# Autodesk Inventor assembly: LeftMecanumDTANewAttachment
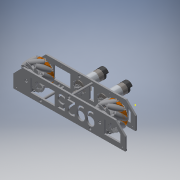
[picture p0: Inventor's stored thumbnail of the model, 180x180]
Saved by Autodesk Inventor 2017 (Build 210142000, 142)
## iProperties
Created: 2017-08-12
Part Number: LeftMecanumDTANewAttachment
Document SubType Name: Assembly
Designer: User
Author: User
## Documents named in this file (7)
- C:\Robotics\CAD\2016-17_CAD\DriveTrain\LeftMecanumDTANewAttachment.iam
- C:\Robotics\CAD\2016-17_CAD\DriveTrain\DrainTrainPlate2.0LeftOutside.iam
- C:\Robotics\CAD\2016-17_CAD\DriveTrain\DriveTrainPlate2.0LeftInside.ipt
- C:\Robotics\CAD\2016-17_CAD\DriveTrain\wheel sub assembly mechanum wheels .iam
- C:\Robotics\CAD\2016-17_CAD\DriveTrain\motor sub assembley.iam
- C:\Robotics\CAD\COTSParts\Tetrix\tetrix-motor-mounts-1.snapshot.1\Tetrex 2pc motor mount.ipt
- C:\Robotics\CAD\2016-17_CAD\DriveTrain\drive train standoff.0002.ipt
## Components (11 placed, 6 different names)
1. DrainTrainPlate2.0LeftOutside:1 [sub-assembly] — Flush:2, Mate:3, Flush:3, Mate:4, Flush:5, Mate:14, Mate:15, Mate:16
2. DriveTrainPlate2.0LeftInside:1 — Mate:2, Flush:4, Mate:5, Flush:6, Mate:6, Mate:7, Mate:8, Mate:10, Mate:11, Mate:12
3. wheel sub assembly mechanum wheels :1 [sub-assembly] — Mate:4, Flush:5, Mate:5, Flush:6, Flush:7
4. wheel sub assembly mechanum wheels :2 [sub-assembly] — Flush:2, Mate:2, Mate:3, Flush:3, Flush:4, Flush:8
5. motor sub assembley:1 [sub-assembly] — Mate:13, Flush:8
6. motor sub assembley:2 [sub-assembly] — Mate:9, Flush:7
7. Tetrex 2pc motor mount:1 — Mate:6, Mate:7, Mate:8, Mate:9
8. Tetrex 2pc motor mount:2 — Mate:10, Mate:11, Mate:12, Mate:13
9. drive train standoff.0002:1 — Mate:14
10. drive train standoff.0002:2 — Mate:15
11. drive train standoff.0002:3 — Mate:16
## Relationships (22: Mate 15, Flush 7)
- Flush:2: DrainTrainPlate2.0LeftOutside:1 ↔ wheel sub assembly mechanum wheels :2
- Mate:2: DriveTrainPlate2.0LeftInside:1 ↔ wheel sub assembly mechanum wheels :2
- Mate:3: DrainTrainPlate2.0LeftOutside:1 ↔ wheel sub assembly mechanum wheels :2
- Flush:3: DrainTrainPlate2.0LeftOutside:1 ↔ wheel sub assembly mechanum wheels :2
- Flush:4: DriveTrainPlate2.0LeftInside:1 ↔ wheel sub assembly mechanum wheels :2
- Mate:4: DrainTrainPlate2.0LeftOutside:1 ↔ wheel sub assembly mechanum wheels :1
- Flush:5: DrainTrainPlate2.0LeftOutside:1 ↔ wheel sub assembly mechanum wheels :1
- Mate:5: DriveTrainPlate2.0LeftInside:1 ↔ wheel sub assembly mechanum wheels :1
- Flush:6: DriveTrainPlate2.0LeftInside:1 ↔ wheel sub assembly mechanum wheels :1
- Mate:6: DriveTrainPlate2.0LeftInside:1 ↔ Tetrex 2pc motor mount:1
- Mate:7: DriveTrainPlate2.0LeftInside:1 ↔ Tetrex 2pc motor mount:1
- Mate:8: DriveTrainPlate2.0LeftInside:1 ↔ Tetrex 2pc motor mount:1
- Mate:9: motor sub assembley:2 ↔ Tetrex 2pc motor mount:1
- Flush:7: wheel sub assembly mechanum wheels :1 ↔ motor sub assembley:2
- Mate:10: DriveTrainPlate2.0LeftInside:1 ↔ Tetrex 2pc motor mount:2
- Mate:11: DriveTrainPlate2.0LeftInside:1 ↔ Tetrex 2pc motor mount:2
- Mate:12: DriveTrainPlate2.0LeftInside:1 ↔ Tetrex 2pc motor mount:2
- Mate:13: motor sub assembley:1 ↔ Tetrex 2pc motor mount:2
- Flush:8: wheel sub assembly mechanum wheels :2 ↔ motor sub assembley:1
- Mate:14: DrainTrainPlate2.0LeftOutside:1 ↔ drive train standoff.0002:1
- Mate:15: DrainTrainPlate2.0LeftOutside:1 ↔ drive train standoff.0002:2
- Mate:16: DrainTrainPlate2.0LeftOutside:1 ↔ drive train standoff.0002:3
